# Autodesk Inventor assembly: Ground_Antenna700mm
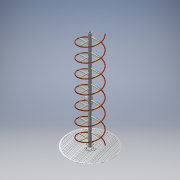
[picture p0: Inventor's stored thumbnail of the model, 180x180]
Saved by Autodesk Inventor 2018 (Build 220112000, 112)
## iProperties
Created: 2018-09-26
Part Number: Ground_Antenna700mm
Document SubType Name: Assembly
Designer: Bradley
Mass: 2554.56 g
Surface Area: 9289.92 cm^2
Volume: 1144.78 cm^3
Density: 2.2315 g/cm^3
Author: Bradley
## Documents named in this file (7)
- C:\Users\Bradley\Documents\GitHub\CougSat1-Hardware\CougSat1-GroundStation\CADModel\Native\Ground_Antenna700mm.iam
- C:\Users\Bradley\Documents\GitHub\CougSat1-Hardware\CougSat1-GroundStation\CADModel\Native\Ground_Antenna700mm_Reflector.ipt
- C:\Users\Bradley\Documents\GitHub\CougSat1-Hardware\CougSat1-GroundStation\CADModel\Native\Ground_Antenna700mm_Helix.ipt
- C:\Users\Bradley\Documents\GitHub\Resources\ComponentModels\Hardware\Piping_Flange_1in.ipt
- C:\Users\Bradley\Documents\GitHub\CougSat1-Hardware\CougSat1-GroundStation\CADModel\Native\Ground_Antenna700mm_Support.ipt
- C:\Users\Bradley\Documents\GitHub\CougSat1-Hardware\CougSat1-GroundStation\CADModel\Native\Ground_Antenna700mm_SupportArm.ipt
- C:\Users\Bradley\Documents\GitHub\Resources\ComponentModels\Hardware\Piping_TeeInline_1in.ipt
## Components (33 placed, 6 different names)
1. Ground_Antenna700mm_Reflector:1 — Flush:1, Insert:1, Insert:2
2. Ground_Antenna700mm_Helix:1 — Mate:1, Flush:1, Mate:5, Angle:1, Mate:9, Mate:10, Mate:12
3. Piping_Flange_1in:1 — Insert:1, Insert:2, Insert:3
4. Ground_Antenna700mm_Support:1 — Insert:3, Mate:2, Mate:3, Mate:6, Mate:7, Mate:8, Mate:14, Mate:15
5. Piping_TeeInline_1in:1 — Mate:15, Mate:16, Mate:17
6. Ground_Antenna700mm_SupportArm:1 — Mate:3, Mate:5, Flush:7, Mate:14
7. Ground_Antenna700mm_SupportArm:2 — Mate:6, Mate:9, Flush:8
8. Ground_Antenna700mm_SupportArm:3 — Mate:7, Mate:10, Mate:11
9. Ground_Antenna700mm_SupportArm:4 — Mate:8, Mate:12, Mate:13
10. Ground_Antenna700mm_SupportArm:5
11. Ground_Antenna700mm_SupportArm:6
12. Ground_Antenna700mm_SupportArm:7
13. Ground_Antenna700mm_SupportArm:8
14. Ground_Antenna700mm_SupportArm:9
15. Ground_Antenna700mm_SupportArm:10
16. Ground_Antenna700mm_SupportArm:11
17. Ground_Antenna700mm_SupportArm:12
18. Ground_Antenna700mm_SupportArm:13
19. Ground_Antenna700mm_SupportArm:14
20. Ground_Antenna700mm_SupportArm:15
21. Ground_Antenna700mm_SupportArm:16
22. Ground_Antenna700mm_SupportArm:17
23. Ground_Antenna700mm_SupportArm:18
24. Ground_Antenna700mm_SupportArm:19
25. Ground_Antenna700mm_SupportArm:20
26. Ground_Antenna700mm_SupportArm:21
27. Ground_Antenna700mm_SupportArm:22
28. Ground_Antenna700mm_SupportArm:23
29. Ground_Antenna700mm_SupportArm:24
30. Ground_Antenna700mm_SupportArm:25
31. Ground_Antenna700mm_SupportArm:26
32. Ground_Antenna700mm_SupportArm:27
33. Ground_Antenna700mm_SupportArm:28
## Component patterns: (7 elements, first: Ground_Antenna700mm_SupportArm:1 + Ground_Antenna700mm_SupportArm:2 + Ground_Antenna700mm_SupportArm:3 + Ground_Antenna700mm_SupportArm:4)
## Relationships (23: Mate 16, Flush 3, Insert 3, Angle 1)
- Mate:1: Ground_Antenna700mm_Helix:1
- Flush:1 (-6.6 mm): Ground_Antenna700mm_Reflector:1 ↔ Ground_Antenna700mm_Helix:1
- Insert:1: Ground_Antenna700mm_Reflector:1 ↔ Piping_Flange_1in:1
- Insert:2: Ground_Antenna700mm_Reflector:1 ↔ Piping_Flange_1in:1
- Insert:3: Piping_Flange_1in:1 ↔ Ground_Antenna700mm_Support:1
- Mate:2: Ground_Antenna700mm_Support:1
- Mate:3: Ground_Antenna700mm_Support:1 ↔ Ground_Antenna700mm_SupportArm:1
- Mate:5 (19.825 mm): Ground_Antenna700mm_Helix:1 ↔ Ground_Antenna700mm_SupportArm:1
- Flush:7: Ground_Antenna700mm_SupportArm:1
- Angle:1 (-45 deg): Ground_Antenna700mm_Helix:1
- Mate:6: Ground_Antenna700mm_Support:1 ↔ Ground_Antenna700mm_SupportArm:2
- Mate:7: Ground_Antenna700mm_Support:1 ↔ Ground_Antenna700mm_SupportArm:3
- Mate:8: Ground_Antenna700mm_Support:1 ↔ Ground_Antenna700mm_SupportArm:4
- Mate:9 (59.475 mm): Ground_Antenna700mm_Helix:1 ↔ Ground_Antenna700mm_SupportArm:2
- Flush:8: Ground_Antenna700mm_SupportArm:2
- Mate:10 (99.125 mm): Ground_Antenna700mm_Helix:1 ↔ Ground_Antenna700mm_SupportArm:3
- Mate:11: Ground_Antenna700mm_SupportArm:3
- Mate:12 (138.775 mm): Ground_Antenna700mm_Helix:1 ↔ Ground_Antenna700mm_SupportArm:4
- Mate:13: Ground_Antenna700mm_SupportArm:4
- Mate:14: Ground_Antenna700mm_Support:1 ↔ Ground_Antenna700mm_SupportArm:1
- Mate:15: Ground_Antenna700mm_Support:1 ↔ Piping_TeeInline_1in:1
- Mate:16 (455.8186 mm): Piping_TeeInline_1in:1
- Mate:17: Piping_TeeInline_1in:1
